# Autodesk Inventor assembly: Motor_Node
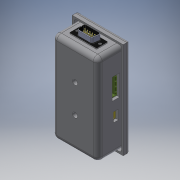
[picture p0: Inventor's stored thumbnail of the model, 180x180]
Saved by Autodesk Inventor 2019 (Build 230136000, 136)
## iProperties
Created: 2019-12-12
Part Number: Motor_Node
Document SubType Name: Assembly
Designer: Jorian Brusind
Author: Jorian Brusind
## Documents named in this file (6)
- C:\Users\Jorian Brusind\Documents\GitHub\ECE44x_Senior_Design\Design files\Delta Robot Arm\Inventor Files\Custom_Delta\Motor_Node.iam
- C:\Users\Jorian Brusind\Documents\GitHub\ECE44x_Senior_Design\Design files\Delta Robot Arm\Inventor Files\Custom_Delta\Motor_Node_box.ipt
- C:\Users\Jorian Brusind\Documents\GitHub\ECE44x_Senior_Design\Design files\Delta Robot Arm\Inventor Files\Custom_Delta\Motor_Node_top.ipt
- C:\Users\Jorian Brusind\Documents\GitHub\ECE44x_Senior_Design\Design files\Delta Robot Arm\Inventor Files\amass-xt30pw-m-_-pcb-solder-1.snapshot.2\XT30.ipt
- C:\Users\Jorian Brusind\Documents\GitHub\ECE44x_Senior_Design\Design files\Delta Robot Arm\Inventor Files\ci32-8-pin-connector-1.snapshot.1\CONNECTOR DB_9_MALE.ipt
- C:\Users\Jorian Brusind\Documents\GitHub\ECE44x_Senior_Design\Design files\Delta Robot Arm\Inventor Files\ENG_CVM_796638-4_C3.3d_stp\c-796638-4-c3-3d.ipt
## Components (6 placed, 5 different names)
1. Motor_Node_box:1 — Mate:3, Mate:4, Mate:5, Mate:6, Mate:7, Mate:8, Mate:9, Mate:11, Mate:12, Mate:13, Mate:14, Mate:15, Mate:16, Mate:17, Mate:18
2. Motor_Node_top:1 — Mate:16, Mate:17, Mate:18
3. XT30:1 — Mate:11, Mate:12, Mate:13
4. CONNECTOR DB_9_MALE:1 — Mate:3, Mate:14, Mate:15
5. CONNECTOR DB_9_MALE:2 — Mate:4, Mate:5, Mate:6
6. c-796638-4-c3-3d:1 — Mate:7, Mate:8, Mate:9
## Relationships (15: Mate 15)
- Mate:3: Motor_Node_box:1 ↔ CONNECTOR DB_9_MALE:1
- Mate:4: Motor_Node_box:1 ↔ CONNECTOR DB_9_MALE:2
- Mate:5: Motor_Node_box:1 ↔ CONNECTOR DB_9_MALE:2
- Mate:6: Motor_Node_box:1 ↔ CONNECTOR DB_9_MALE:2
- Mate:7 (0.5 mm): Motor_Node_box:1 ↔ c-796638-4-c3-3d:1
- Mate:8 (0.5 mm): Motor_Node_box:1 ↔ c-796638-4-c3-3d:1
- Mate:9: Motor_Node_box:1 ↔ c-796638-4-c3-3d:1
- Mate:11 (0.25 mm): Motor_Node_box:1 ↔ XT30:1
- Mate:12: Motor_Node_box:1 ↔ XT30:1
- Mate:13 (0.25 mm): Motor_Node_box:1 ↔ XT30:1
- Mate:14: Motor_Node_box:1 ↔ CONNECTOR DB_9_MALE:1
- Mate:15: Motor_Node_box:1 ↔ CONNECTOR DB_9_MALE:1
- Mate:16: Motor_Node_box:1 ↔ Motor_Node_top:1
- Mate:17: Motor_Node_box:1 ↔ Motor_Node_top:1
- Mate:18: Motor_Node_box:1 ↔ Motor_Node_top:1
